# Autodesk Inventor assembly: Tattu 850mah 4S
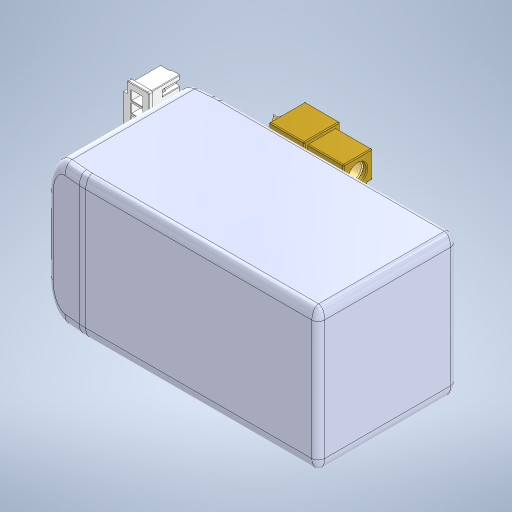
[picture p0: Inventor's stored thumbnail of the model, 512x512]
Saved by Autodesk Inventor 2023.1 (Build 271208000, 208)
## iProperties
Created: 2022-12-23
Part Number: Tattu 850mah 4S
Document SubType Name: Assembly
Designer: Nathan Cai
Author: Nathan Cai
## Documents named in this file (4)
- E:\Documents\Inventor\Law - V1.0\Tattu 4S 650mah\Tattu 850mah 4S.iam
- E:\Documents\Inventor\Law - V1.0\Tattu 4S 650mah\FUNDA 13.ipt
- E:\Documents\Inventor\Law - V1.0\Tattu 4S 650mah\XT60 Buchse.ipt
- E:\Documents\Inventor\Law - V1.0\Tattu 4S 650mah\JST XHP-4.ipt
## Components (3 placed, 3 different names)
1. FUNDA 13:1 — Mate:1, Flush:1, Flush:2, Mate:2, Flush:3
2. XT60 Buchse:1 — Mate:1, Flush:1
3. JST XHP-4:1 — Flush:2, Mate:2, Flush:3
## Relationships (5: Flush 3, Mate 2)
- Mate:1: FUNDA 13:1 ↔ XT60 Buchse:1
- Flush:1: FUNDA 13:1 ↔ XT60 Buchse:1
- Flush:2: FUNDA 13:1 ↔ JST XHP-4:1
- Mate:2: FUNDA 13:1 ↔ JST XHP-4:1
- Flush:3: FUNDA 13:1 ↔ JST XHP-4:1
